# Autodesk Inventor assembly: clamp
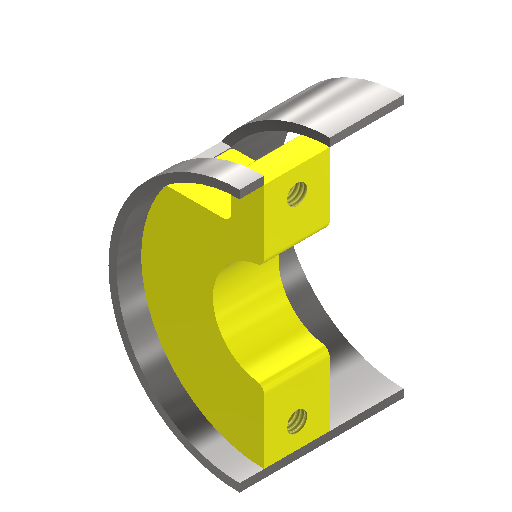
[picture p0: Inventor's stored thumbnail of the model, 512x512]
Saved by Autodesk Inventor 2026 (Build 300175050, 175E)
## iProperties
Created: 2025-10-23
Part Number: clamp
Document SubType Name: Assembly
Designer: jin20
Author: jin20
## Documents named in this file (3)
- C:\Users\jin20\Documents\装置CAD\SpectroscopySystem\Probe\clamp.iam
- C:\Users\jin20\Documents\装置CAD\SpectroscopySystem\Probe\clamp-ring.ipt
- C:\Users\jin20\Documents\装置CAD\SpectroscopySystem\Probe\cover-pipe.ipt
## Components (2 placed, 2 different names)
1. clamp-ring:1 — 挿入:1
2. cover-pipe:1 — 挿入:1
## Relationships (1: Insert 1)
- 挿入:1 [Insert] (-11 mm): clamp-ring:1 ↔ cover-pipe:1
